# Autodesk Inventor assembly: Wasabi
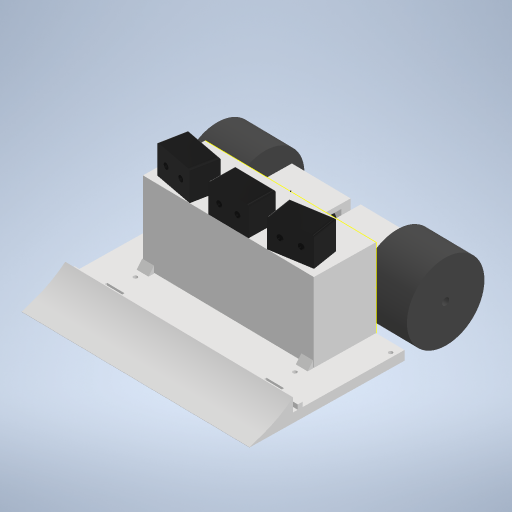
[picture p0: Inventor's stored thumbnail of the model, 512x512]
Saved by Autodesk Inventor 2024 (Build 280153000, 153)
## iProperties
Created: 2023-10-20
Part Number: Wasabi
Document SubType Name: Assembly
Designer: kdcao
Author: kdcao
## Documents named in this file (8)
- C:\Users\kdcao\Downloads\Wasabi\Wasabi.iam
- C:\Users\kdcao\Downloads\Wasabi\Wasabi\Body.ipt
- C:\Users\kdcao\Downloads\Wasabi\battery.ipt
- C:\Users\kdcao\Downloads\Wasabi\qtr-1a-reflectance-sensor.ipt
- C:\Users\kdcao\Downloads\Wasabi\Wasabi\wheel.ipt
- C:\Users\kdcao\Downloads\Wasabi\micro-metal-gearmotor-standard\micro-metal-gearmotor-standard.ipt
- C:\Users\kdcao\Downloads\Wasabi\board.ipt
- C:\Users\kdcao\Downloads\Wasabi\Wasabi\IR sensor.ipt
## Components (12 placed, 7 different names)
1. Body:1 — Angle:1, Flush:3, Mate:3, Flush:4, Tangent:1, Tangent:2, Flush:5, Mate:5, Flush:6, Tangent:3, Tangent:4, Mate:7, Mate:8, Flush:7, Angle:2, Mate:13, Mate:14, Angle:3, Mate:15, Mate:17, Mate:18, Rigid:2, Rigid:3
2. battery:1 — Angle:1, Flush:3, Mate:3, Flush:4, Mate:6, Mate:9, Mate:11, Mate:12
3. qtr-1a-reflectance-sensor:1 — Rigid:3
4. qtr-1a-reflectance-sensor:2 — Rigid:2
5. wheel:2 — Tangent:1, Tangent:2, Flush:5, Cylindrical:1, Mate:4
6. micro-metal-gearmotor-standard:2 — Cylindrical:1, Mate:4
7. wheel:3 — Rotational:1, Flush:6, Tangent:3, Tangent:4
8. micro-metal-gearmotor-standard:3 — Mate:5, Rotational:1
9. board:1 — Mate:6, Mate:7, Mate:8, Mate:10
10. IR sensor:1 — Mate:9, Flush:7, Mate:10, Mate:16
11. IR sensor:2 — Mate:11, Angle:2, Mate:13, Mate:14, Mate:18
12. IR sensor:3 — Mate:12, Angle:3, Mate:15, Mate:16, Mate:17
## Relationships (32: Mate 16, Flush 5, Tangent 4, Angle 3, WeldJoint 2, CylindricalJoint 1, RevoluteJoint 1)
- Angle:1 (0 deg): Body:1 ↔ battery:1
- Flush:3: Body:1 ↔ battery:1
- Mate:3: Body:1 ↔ battery:1
- Flush:4: Body:1 ↔ battery:1
- Tangent:1 (1 mm): Body:1 ↔ wheel:2
- Tangent:2 (1 mm): Body:1 ↔ wheel:2
- Flush:5: Body:1 ↔ wheel:2
- Cylindrical:1: wheel:2 ↔ micro-metal-gearmotor-standard:2
- Mate:4: wheel:2 ↔ micro-metal-gearmotor-standard:2
- Mate:5: Body:1 ↔ micro-metal-gearmotor-standard:3
- Rotational:1 [RevoluteJoint]: wheel:3 ↔ micro-metal-gearmotor-standard:3
- Flush:6: Body:1 ↔ wheel:3
- Tangent:3 (1 mm): Body:1 ↔ wheel:3
- Tangent:4 (1 mm): Body:1 ↔ wheel:3
- Mate:6 (1 mm): battery:1 ↔ board:1
- Mate:7: Body:1 ↔ board:1
- Mate:8 (3 mm): Body:1 ↔ board:1
- Mate:9: battery:1 ↔ IR sensor:1
- Flush:7: Body:1 ↔ IR sensor:1
- Mate:10 (12 mm): board:1 ↔ IR sensor:1
- Mate:11: battery:1 ↔ IR sensor:2
- Mate:12: battery:1 ↔ IR sensor:3
- Angle:2 (10 deg): Body:1 ↔ IR sensor:2
- Mate:13 (-15 mm): Body:1 ↔ IR sensor:2
- Mate:14: Body:1 ↔ IR sensor:2
- Angle:3 (-10 deg): Body:1 ↔ IR sensor:3
- Mate:15 (15 mm): Body:1 ↔ IR sensor:3
- Mate:16: IR sensor:1 ↔ IR sensor:3
- Mate:17: Body:1 ↔ IR sensor:3
- Mate:18: Body:1 ↔ IR sensor:2
- Rigid:2 [WeldJoint]: Body:1 ↔ qtr-1a-reflectance-sensor:2
- Rigid:3 [WeldJoint]: Body:1 ↔ qtr-1a-reflectance-sensor:1
